# Autodesk Inventor assembly: XEndLeft
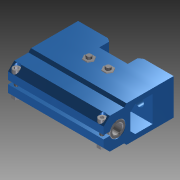
[picture p0: Inventor's stored thumbnail of the model, 180x180]
Saved by Autodesk Inventor 2015 (Build 190159000, 159)
## iProperties
Created: 2014-08-16
Part Number: XEndLeft
Document SubType Name: Assembly
Designer: Jack
Author: Jack
## Documents named in this file (13)
- C:\Users\Jack\ownCloud\Projects\CoreXY\InventorModel\XAxis\DualE3DXEnd\XEndLeft.iam
- C:\Users\Jack\ownCloud\Projects\CoreXY\InventorModel\XAxis\DualE3DXEnd\XEnd.ipt
- C:\Users\Jack\ownCloud\Projects\CoreXY\InventorModel\Hardware\Nuts\Nut3.ipt
- C:\Users\Jack\ownCloud\Projects\CoreXY\InventorModel\Hardware\Bolts\SHCS\SHCS3\SHCS3x18.ipt
- C:\Users\Jack\ownCloud\Projects\CoreXY\InventorModel\Hardware\Bolts\SHCS\SHCS4\SHCS4x30.ipt
- C:\Users\Jack\ownCloud\Projects\CoreXY\InventorModel\Hardware\Nuts\Nut4.ipt
- C:\Users\Jack\ownCloud\Projects\CoreXY\InventorModel\Hardware\Bearing\BearingRadialBall\BearingRadialBallF624zz.ipt
- C:\Users\Jack\ownCloud\Projects\CoreXY\InventorModel\Hardware\Wahsers\M4Washer.ipt
- C:\Users\Jack\ownCloud\Projects\CoreXY\InventorModel\Hardware\Bolts\SHCS\SHCS3\SHCS3x8.ipt
- C:\Users\Jack\ownCloud\Projects\CoreXY\InventorModel\XAxis\DualE3DXEnd\XAxisBearingSpacer.ipt
- C:\Users\Jack\ownCloud\Projects\CoreXY\InventorModel\Hardware\Bearing\BearingLinear\BearingLinearLMK8.ipt
- C:\Users\Jack\ownCloud\Projects\CoreXY\InventorModel\Hardware\Belt\GT2Idler.iam
- C:\Users\Jack\ownCloud\Projects\CoreXY\InventorModel\XAxis\DualE3DXEnd\XAxisBeltIdlerSpacer.ipt
## Components (24 placed, 12 different names)
1. XEnd:1 — Mate:5, Mate:6, Mate:7, Mate:8, Mate:9, Angle:1, Angle:2, Mate:10, Mate:11, Mate:13, Mate:15, Mate:16, Mate:17, Mate:18, Mate:19, Angle:3, Angle:4, Mate:22, Mate:23, Mate:39, Mate:40, Mate:41, Angle:5, Angle:6, Mate:44, Mate:45, Mate:54, Mate:55, Flush:3, Flush:4, Mate:56, Mate:62
2. XAxisBearingSpacer:2 — Mate:51, Mate:52
3. BearingLinearLMK8:1 — Mate:55, Flush:4
4. BearingLinearLMK8:2 — Mate:54, Flush:3
5. GT2Idler:1 [sub-assembly] — Mate:58, Mate:59, Mate:60
6. XAxisBeltIdlerSpacer:1 — Mate:61, Mate:62
7. BearingRadialBallF624zz:3
8. BearingRadialBallF624zz:4
9. M4Washer:4 — Mate:38, Mate:52
10. M4Washer:3 — Mate:39
11. M4Washer:2 — Mate:30, Mate:56, Mate:59
12. M4Washer:1 — Mate:57, Mate:60
13. Nut4:2 — Mate:21, Angle:4, Mate:23
14. Nut4:1 — Mate:20, Angle:3, Mate:22
15. SHCS4x30:2 — Mate:17, Mate:18, Mate:20, Mate:38, Mate:51
16. SHCS4x30:1 — Mate:16, Mate:19, Mate:21, Mate:30, Mate:57, Mate:58, Mate:61
17. Nut3:3 — Mate:43, Angle:6, Mate:45, Flush:1
18. Nut3:4 — Mate:42, Angle:5, Mate:44, Flush:2
19. SHCS3x8:1 — Mate:40, Mate:42, Flush:2
20. SHCS3x8:2 — Mate:41, Mate:43, Flush:1
21. SHCS3x18:2 — Mate:14, Mate:15
22. SHCS3x18:1 — Mate:12, Mate:13
23. Nut3:2 — Mate:8, Angle:1, Mate:11, Mate:12
24. Nut3:1 — Mate:9, Angle:2, Mate:10, Mate:14
## Relationships (55: Mate 45, Angle 6, Flush 4)
- Mate:5: XEnd:1
- Mate:6: XEnd:1
- Mate:7: XEnd:1
- Mate:8: XEnd:1 ↔ Nut3:2
- Mate:9: XEnd:1 ↔ Nut3:1
- Angle:1 (0 deg): XEnd:1 ↔ Nut3:2
- Angle:2 (0 deg): XEnd:1 ↔ Nut3:1
- Mate:10: XEnd:1 ↔ Nut3:1
- Mate:11: XEnd:1 ↔ Nut3:2
- Mate:12: SHCS3x18:1 ↔ Nut3:2
- Mate:13: XEnd:1 ↔ SHCS3x18:1
- Mate:14: SHCS3x18:2 ↔ Nut3:1
- Mate:15: XEnd:1 ↔ SHCS3x18:2
- Mate:16: XEnd:1 ↔ SHCS4x30:1
- Mate:17: XEnd:1 ↔ SHCS4x30:2
- Mate:18: XEnd:1 ↔ SHCS4x30:2
- Mate:19: XEnd:1 ↔ SHCS4x30:1
- Mate:20: Nut4:1 ↔ SHCS4x30:2
- Mate:21: Nut4:2 ↔ SHCS4x30:1
- Angle:3 (0 deg): XEnd:1 ↔ Nut4:1
- Angle:4 (0 deg): XEnd:1 ↔ Nut4:2
- Mate:22: XEnd:1 ↔ Nut4:1
- Mate:23: XEnd:1 ↔ Nut4:2
- Mate:30: M4Washer:2 ↔ SHCS4x30:1
- [Mate]: BearingRadialBallF624zz:3 ↔ BearingRadialBallF624zz:4
- [Mate]: BearingRadialBallF624zz:3 ↔ BearingRadialBallF624zz:4
- [Mate]: BearingRadialBallF624zz:3 ↔ M4Washer:3
- [Mate]: BearingRadialBallF624zz:3 ↔ M4Washer:3
- [Mate]: BearingRadialBallF624zz:4 ↔ M4Washer:4
- [Mate]: BearingRadialBallF624zz:4 ↔ M4Washer:4
- Mate:38: M4Washer:4 ↔ SHCS4x30:2
- Mate:39: XEnd:1 ↔ M4Washer:3
- Mate:40: XEnd:1 ↔ SHCS3x8:1
- Mate:41: XEnd:1 ↔ SHCS3x8:2
- Mate:42: Nut3:4 ↔ SHCS3x8:1
- Mate:43: Nut3:3 ↔ SHCS3x8:2
- Angle:5 (0 deg): XEnd:1 ↔ Nut3:4
- Angle:6 (0 deg): XEnd:1 ↔ Nut3:3
- Mate:44: XEnd:1 ↔ Nut3:4
- Mate:45: XEnd:1 ↔ Nut3:3
- Flush:1 (-0.5 mm): Nut3:3 ↔ SHCS3x8:2
- Flush:2 (-0.5 mm): Nut3:4 ↔ SHCS3x8:1
- Mate:51: XAxisBearingSpacer:2 ↔ SHCS4x30:2
- Mate:52: XAxisBearingSpacer:2 ↔ M4Washer:4
- Mate:54: XEnd:1 ↔ BearingLinearLMK8:2
- Mate:55: XEnd:1 ↔ BearingLinearLMK8:1
- Flush:3: XEnd:1 ↔ BearingLinearLMK8:2
- Flush:4: XEnd:1 ↔ BearingLinearLMK8:1
- Mate:56: XEnd:1 ↔ M4Washer:2
- Mate:57: M4Washer:1 ↔ SHCS4x30:1
- Mate:58: GT2Idler:1 ↔ SHCS4x30:1
- Mate:59: GT2Idler:1 ↔ M4Washer:2
- Mate:60: GT2Idler:1 ↔ M4Washer:1
- Mate:61: XAxisBeltIdlerSpacer:1 ↔ SHCS4x30:1
- Mate:62: XEnd:1 ↔ XAxisBeltIdlerSpacer:1
## Named parameters: d35_d44 = 0 mm, d36_d45 = 0 mm, d37_d46 = 0 mm, d38_d47 = 0 mm, d39_d48 = 0 mm, d40_d49 = 0 mm
